# Autodesk Inventor assembly: modularRICHFrame
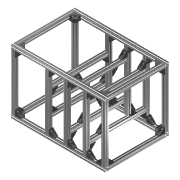
[picture p0: Inventor's stored thumbnail of the model, 180x180]
Saved by Autodesk Inventor 2018.2 (Build 222227000, 227)
## iProperties
Created: 2016-04-02
Part Number: modularRICHFrame
Document SubType Name: Assembly
Designer: sawai
Author: sawai
## Documents named in this file (4)
- C:\Users\sawaiz\OneDrive\projects\modularRICHFrame\modularRICHFrame.iam
- C:\Users\sawaiz\OneDrive\projects\modularRICHFrame\frame\frame.iam
- C:\Users\sawaiz\OneDrive\projects\modularRICHFrame\frame\richHolder.iam
- C:\Users\sawaiz\OneDrive\projects\modularRICHFrame\frame\richHolderSuppourt.iam
## Components (4 placed, 3 different names)
1. frame:1 [sub-assembly] — Mate:1, Flush:1, Flush:2, Mate:2, Mate:3, Flush:3, Flush:4
2. richHolder:1 [sub-assembly] — Mate:1, Flush:1, Flush:4, Flush:5
3. richHolder:2 [sub-assembly] — Flush:2, Mate:2, Flush:5, Flush:6
4. richHolderSuppourt:1 [sub-assembly] — Mate:3, Flush:3, Flush:6
## Relationships (9: Flush 6, Mate 3)
- Mate:1: frame:1 ↔ richHolder:1
- Flush:1: frame:1 ↔ richHolder:1
- Flush:2: frame:1 ↔ richHolder:2
- Mate:2: frame:1 ↔ richHolder:2
- Mate:3: frame:1 ↔ richHolderSuppourt:1
- Flush:3: frame:1 ↔ richHolderSuppourt:1
- Flush:4 (-100 mm): frame:1 ↔ richHolder:1
- Flush:5 (-100 mm): richHolder:1 ↔ richHolder:2
- Flush:6 (-100 mm): richHolder:2 ↔ richHolderSuppourt:1
